# Autodesk Inventor assembly: XPulleySupport
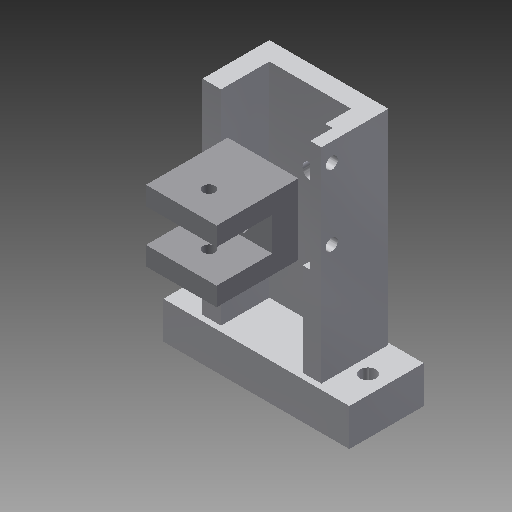
[picture p0: Inventor's stored thumbnail of the model, 512x512]
Saved by Autodesk Inventor 2019 (Build 230136000, 136)
## iProperties
Created: 2019-08-19
Part Number: XPulleySupport
Document SubType Name: Assembly
Designer: Bruno
Mass: 26.4092 g
Surface Area: 120.787 cm^2
Volume: 25.2032 cm^3
Density: 1.04785 g/cm^3
Author: Bruno
## Documents named in this file (3)
- C:\Users\Bruno\Stuff\Ajedrez2\XPulleySupport.iam
- C:\Users\Bruno\Stuff\Ajedrez2\XPulleySupportBase.ipt
- C:\Users\Bruno\Stuff\Ajedrez2\XPulleySupportHolder.ipt
## Components (2 placed, 2 different names)
1. XPulleySupportBase:1 — Cylindrical:1, Angle:1
2. XPulleySupportHolder:1 — Cylindrical:1, Angle:1
## Relationships (2: CylindricalJoint 1, Angle 1)
- Cylindrical:1: XPulleySupportBase:1 ↔ XPulleySupportHolder:1
- Angle:1 (0 deg): XPulleySupportBase:1 ↔ XPulleySupportHolder:1
